# Autodesk Inventor assembly: doorLockAssembly_V2
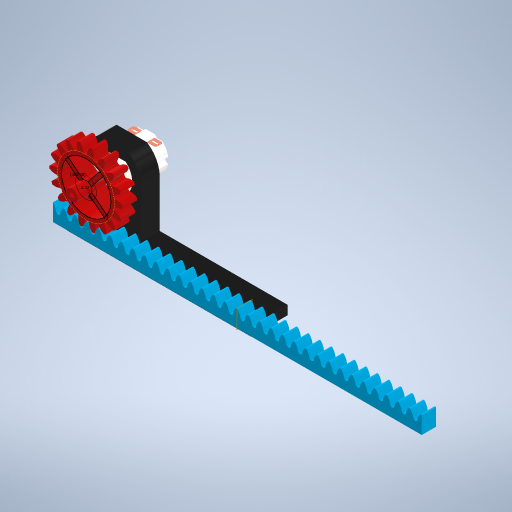
[picture p0: Inventor's stored thumbnail of the model, 512x512]
Saved by Autodesk Inventor 2023 (Build 270158000, 158)
## iProperties
Created: 2022-11-21
Part Number: doorLockAssembly_V2
Document SubType Name: Assembly
Designer: shrey
Author: shrey
## Documents named in this file (6)
- D:\Inventor Projects\Door Lock\V2\doorLockAssembly_V2.iam
- D:\Inventor Projects\Door Lock\V2\doorLockAssembly_V2\Design Accelerator\Spur Gears1.iam
- D:\Inventor Projects\Door Lock\V2\gear_V2.ipt
- D:\Inventor Projects\Door Lock\V2\pinion_V2.ipt
- D:\Inventor Projects\Door Lock\motor.ipt
- D:\Inventor Projects\Door Lock\V2\tempHolder_V2.ipt
## Components (5 placed, 5 different names)
1. Spur Gears:1 [sub-assembly]
2. gear_V2:1 — Mate:1, Flush:1, Flush:4, Rotation/Translation:1
3. pinion_V2:1 — Flush:4, Mate:3, Rotation/Translation:1
4. motor:1 — Mate:2, Flush:2, Flush:3
5. tempHolder_V2:1
## Relationships (9: Flush 5, Mate 3, RelateRotateTranslate 1)
- Mate:1: gear_V2:1
- Flush:1: gear_V2:1
- Mate:2: motor:1
- Flush:2: motor:1
- Flush:3: motor:1
- Flush:4: gear_V2:1 ↔ pinion_V2:1
- Mate:3 (-18 mm): pinion_V2:1
- Rotation/Translation:1 [RelateRotateTranslate] (113.0973 mm): gear_V2:1 ↔ pinion_V2:1
- Flush:5 (-15 mm)
